# Autodesk Inventor assembly: atarasiiude
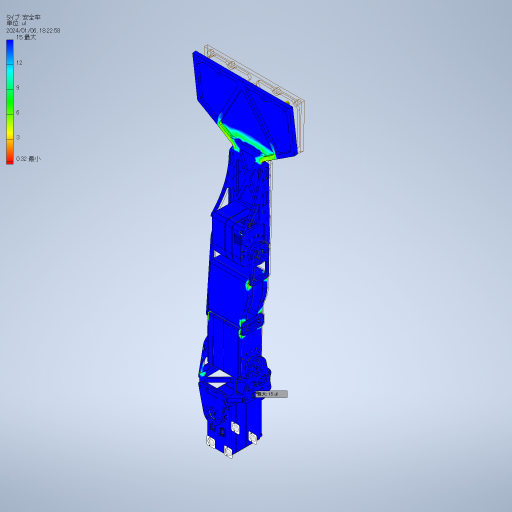
[picture p0: Inventor's stored thumbnail of the model, 512x512]
Saved by Autodesk Inventor 2024 (Build 280153000, 153)
## iProperties
Created: 2024-01-03
Part Number: atarasiiude
Document SubType Name: Assembly
Designer: right
Mass: 160.562 g
Surface Area: 631.955 cm^2
Volume: 103.154 cm^3
Density: 1.55653 g/cm^3
Author: right
## Documents named in this file (19)
- C:\Users\right\OneDrive\ドキュメント\Inventor\V2二足Light＿仮\atarasiiude.iam
- C:\Users\right\OneDrive\ドキュメント\Inventor\V2二足Light＿仮\KRS2500_scale3.ipt
- C:\Users\right\OneDrive\ドキュメント\Inventor\V2二足Light＿仮\02159_SmallFreeHornC_MIR2.ipt
- C:\Users\right\OneDrive\ドキュメント\Inventor\V2二足Light＿仮\02157_SmallDiameterHornB_MIR1.ipt
- C:\Users\right\OneDrive\ドキュメント\Inventor\V2二足Light＿仮\kata_new.ipt
- C:\Users\right\OneDrive\ドキュメント\Inventor\V2二足Light＿仮\new_kata_3.ipt
- C:\Users\right\OneDrive\ドキュメント\Inventor\V2二足Light＿仮\kata_new_1.5.ipt
- C:\Users\right\OneDrive\ドキュメント\Inventor\V2二足Light＿仮\tesaki_arata.iam
- C:\Users\right\OneDrive\ドキュメント\Inventor\V2二足Light＿仮\3204ude.ipt
- C:\Users\right\OneDrive\ドキュメント\Inventor\V2二足Light＿仮\newnewude.ipt
- C:\Users\right\OneDrive\ドキュメント\Inventor\V2二足Light＿仮\hera_porika2.ipt
- C:\Users\right\OneDrive\ドキュメント\Inventor\V2二足Light＿仮\3dprintsuzikai.ipt
- C:\Users\right\OneDrive\ドキュメント\Inventor\V2二足Light＿仮\newnewude_2.ipt
- C:\Users\right\OneDrive\ドキュメント\Inventor\V2二足Light＿仮\atarasiiude\AIP\FEA\ekh2g6mdc.fins
- C:\Users\right\OneDrive\ドキュメント\Inventor\V2二足Light＿仮\atarasiiude\AIP\FEA\ekh2g6mdc.fsat
- C:\Users\right\OneDrive\ドキュメント\Inventor\V2二足Light＿仮\atarasiiude\AIP\FEA\ekh2g6mdc.ftes
- C:\Users\right\OneDrive\ドキュメント\Inventor\V2二足Light＿仮\atarasiiude\AIP\FEA\ekh2g6mdc.fwiz
- C:\Users\right\OneDrive\ドキュメント\Inventor\V2二足Light＿仮\atarasiiude\AIP\FEA\ekh2g6mjk.fmsh
- C:\Users\right\OneDrive\ドキュメント\Inventor\V2二足Light＿仮\atarasiiude\AIP\FEA\ekh2g6mjl.fres
## Components (19 placed, 12 different names)
1. KRS2500_scale3:1 — 角度:3
2. 02159_SmallFreeHornC_MIR2:1
3. 02157_SmallDiameterHornB_MIR1:1
4. kata_new:1
5. new_kata_3:1 — 角度:3
6. kata_new:2
7. kata_new_1.5:1
8. kata_new_1.5:2
9. KRS2500_scale3:2 — 挿入:35, 挿入:36, 挿入:43
10. 02159_SmallFreeHornC_MIR2:2
11. 02157_SmallDiameterHornB_MIR1:2
12. 02159_SmallFreeHornC_MIR2:3 — 挿入:50
13. tesaki_arata:1 [sub-assembly] — 挿入:33, 挿入:34, 挿入:50
14. hera_porika2:1 — 挿入:33
15. 02157_SmallDiameterHornB_MIR1:3 — 挿入:34, 挿入:40, 挿入:41
16. newnewude:1 — 挿入:43, 挿入:48, 挿入:49
17. 3204ude:1 — 挿入:35, 挿入:36, 挿入:40, 挿入:41, フラッシュ:3, 挿入:44, 挿入:45
18. 3dprintsuzikai:1 — フラッシュ:3, 挿入:44, 挿入:45, 挿入:48, 挿入:49, フラッシュ:4
19. newnewude_2:1 — フラッシュ:4
## Relationships (37: Insert 32, Flush 4, Angle 1)
- [Insert]: KRS2500_scale3:1 ↔ 02159_SmallFreeHornC_MIR2:1
- [Insert]: KRS2500_scale3:1 ↔ 02157_SmallDiameterHornB_MIR1:1
- [Flush]: 02157_SmallDiameterHornB_MIR1:1 ↔ kata_new:1
- [Insert]: 02157_SmallDiameterHornB_MIR1:1 ↔ kata_new:1
- [Insert]: 02157_SmallDiameterHornB_MIR1:1 ↔ kata_new:1
- [Flush]: kata_new:1 ↔ new_kata_3:1
- [Insert]: 02159_SmallFreeHornC_MIR2:1 ↔ kata_new:2
- [Insert]: 02159_SmallFreeHornC_MIR2:1 ↔ kata_new:2
- [Insert]: new_kata_3:1 ↔ kata_new:2
- [Insert]: kata_new:1 ↔ new_kata_3:1
- [Insert]: kata_new:1 ↔ new_kata_3:1
- [Insert]: new_kata_3:1 ↔ kata_new:2
- [Insert]: new_kata_3:1 ↔ kata_new_1.5:1
- [Insert]: new_kata_3:1 ↔ kata_new_1.5:1
- [Insert]: new_kata_3:1 ↔ kata_new_1.5:2
- [Insert]: new_kata_3:1 ↔ kata_new_1.5:2
- [Insert]: KRS2500_scale3:2 ↔ 02159_SmallFreeHornC_MIR2:2
- [Insert]: KRS2500_scale3:2 ↔ 02157_SmallDiameterHornB_MIR1:2
- [Insert]: kata_new_1.5:1 ↔ 02157_SmallDiameterHornB_MIR1:2
- [Insert]: kata_new_1.5:1 ↔ 02157_SmallDiameterHornB_MIR1:2
- [Insert]: kata_new_1.5:2 ↔ 02159_SmallFreeHornC_MIR2:2
- [Insert]: kata_new_1.5:2 ↔ 02159_SmallFreeHornC_MIR2:2
- 角度:3 [Angle] (0 deg): KRS2500_scale3:1 ↔ new_kata_3:1
- 挿入:33 [Insert]: tesaki_arata:1 ↔ hera_porika2:1
- 挿入:34 [Insert]: tesaki_arata:1 ↔ 02157_SmallDiameterHornB_MIR1:3
- 挿入:35 [Insert]: KRS2500_scale3:2 ↔ 3204ude:1
- 挿入:36 [Insert]: KRS2500_scale3:2 ↔ 3204ude:1
- 挿入:40 [Insert]: 02157_SmallDiameterHornB_MIR1:3 ↔ 3204ude:1
- 挿入:41 [Insert]: 02157_SmallDiameterHornB_MIR1:3 ↔ 3204ude:1
- 挿入:43 [Insert]: KRS2500_scale3:2 ↔ newnewude:1
- フラッシュ:3 [Flush]: 3204ude:1 ↔ 3dprintsuzikai:1
- 挿入:44 [Insert]: 3204ude:1 ↔ 3dprintsuzikai:1
- 挿入:45 [Insert]: 3204ude:1 ↔ 3dprintsuzikai:1
- 挿入:48 [Insert]: newnewude:1 ↔ 3dprintsuzikai:1
- 挿入:49 [Insert]: newnewude:1 ↔ 3dprintsuzikai:1
- 挿入:50 [Insert]: 02159_SmallFreeHornC_MIR2:3 ↔ tesaki_arata:1
- フラッシュ:4 [Flush]: 3dprintsuzikai:1 ↔ newnewude_2:1
## Named parameters: d20_d1 = 0 mm, d21_d0 = 0 mm, d6_d22 = 0 mm, sa_0 = 980
note: some values were not read from the file. Shown as the stored number, unit unknown: "sa_0".
